# Autodesk Inventor assembly: mutterOgSkrue
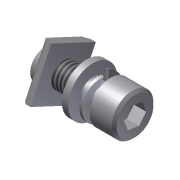
[picture p0: Inventor's stored thumbnail of the model, 180x180]
Saved by Autodesk Inventor 2014 SP1 (Build 180222100, 222)
## iProperties
Created: 2015-02-04
Part Number: mutterOgSkrue
Document SubType Name: Assembly
Designer: Simen
Author: Simen
## Documents named in this file (3)
- C:\Users\Simen\Documents\git\Eit\skjellet\mutterOgSkrue.iam
- C:\Users\Simen\Documents\git\Eit\skjellet\HNTTBS5_5.ipt
- C:\Users\Simen\Documents\git\Eit\skjellet\HCBST5_12.iam
## Components (2 placed, 2 different names)
1. HCBST5-12:1 [sub-assembly]
2. HNTTBS5-5:1
## Relationships (1: Mate 1)
- [Mate]: HCBST5-12:1 ↔ HNTTBS5-5:1
